# Autodesk Inventor assembly: V1Towers
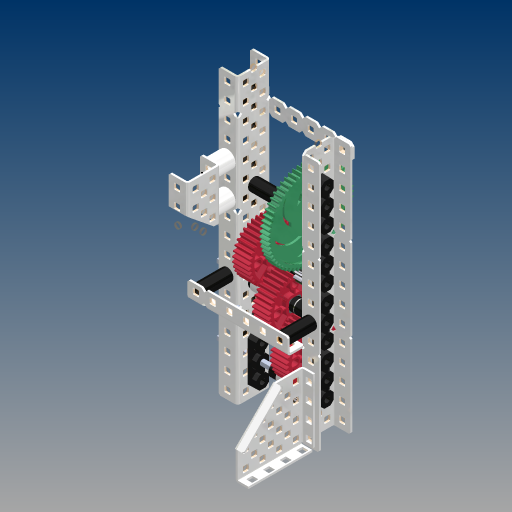
[picture p0: Inventor's stored thumbnail of the model, 512x512]
Saved by Autodesk Inventor 2023 (Build 270158000, 158)
## iProperties
Created: 2023-07-20
Part Number: V1Towers
Document SubType Name: Assembly
Designer: eddie
Author: eddie
## Documents named in this file (26)
- C:\Users\eddie\Documents\81208X-Over-Under-CAD\V1\V1Towers.iam
- C:\Users\eddie\Documents\81208X-Over-Under-CAD\VEX-CAD-Inventor-1.4.0\Structure\C Channel\Aluminum 1x2x1\Alu C 1x2x1x15.ipt
- C:\Users\eddie\Documents\81208X-Over-Under-CAD\VEX-CAD-Inventor-1.4.0\Structure\C Channel\Aluminum 1x2x1\Alu C 1x2x1x17.ipt
- C:\Users\eddie\Documents\81208X-Over-Under-CAD\VEX-CAD-Inventor-1.4.0\Structure\Plate\Aluminum\Alu Plate 1x6.ipt
- C:\Users\eddie\Documents\81208X-Over-Under-CAD\VEX-CAD-Inventor-1.4.0\Motion\Spacers\Spacer Nylon .375 OD\NSpacer .375 OD x .375.ipt
- C:\Users\eddie\Documents\81208X-Over-Under-CAD\VEX-CAD-Inventor-1.4.0\Motion\Spacers\Spacer Nylon .375 OD.ipt
- C:\Users\eddie\Documents\81208X-Over-Under-CAD\VEX-CAD-Inventor-1.4.0\Motion\Spacers\Spacer Nylon .375 OD\NSpacer .375 OD x .500.ipt
- C:\Users\eddie\Documents\81208X-Over-Under-CAD\VEX-CAD-Inventor-1.4.0\Structure\Angle\Aluminum\1x1\Alu Angle 1x1x6.ipt
- C:\Users\eddie\Documents\81208X-Over-Under-CAD\VEX-CAD-Inventor-1.4.0\Motion\Spacers\Spacer Nylon .500 OD\NSpacer White .500 OD x .500.ipt
- C:\Users\eddie\Documents\81208X-Over-Under-CAD\VEX-CAD-Inventor-1.4.0\Motion\Spacers\Spacer Nylon .500 OD.ipt
- C:\Users\eddie\Documents\81208X-Over-Under-CAD\Custom-parts\3x2 channel triangular slice.ipt
- C:\Users\eddie\Documents\81208X-Over-Under-CAD\VEX-CAD-Inventor-1.4.0\Motion\Shaft LS\Bearing Flat.ipt
- C:\Users\eddie\Documents\81208X-Over-Under-CAD\VEX-CAD-Inventor-1.4.0\Structure\Hardware\Nut Alu.ipt
- C:\Users\eddie\Documents\81208X-Over-Under-CAD\VEX-CAD-Inventor-1.4.0\Motion\Gears\HS Gear\HS 12T Gear, Circle.iam
- C:\Users\eddie\Documents\81208X-Over-Under-CAD\VEX-CAD-Inventor-1.4.0\Motion\Gears\HS Gear.iam
- C:\Users\eddie\Documents\81208X-Over-Under-CAD\VEX-CAD-Inventor-1.4.0\Motion\Shaft LS\Shaft LS\Shaft LS 3.0.ipt
- C:\Users\eddie\Documents\81208X-Over-Under-CAD\VEX-CAD-Inventor-1.4.0\Motion\Shaft LS\Shaft LS.ipt
- C:\Users\eddie\Documents\81208X-Over-Under-CAD\Custom-parts\Shaft Collar.ipt
- C:\Users\eddie\Documents\81208X-Over-Under-CAD\VEX-CAD-Inventor-1.4.0\Motion\Gears\LS 12T Gear Steel.ipt
- C:\Users\eddie\Documents\81208X-Over-Under-CAD\VEX-CAD-Inventor-1.4.0\Motion\Spacers\Spacer Nylon .375 OD\NSpacer .375 OD x .125.ipt
- C:\Users\eddie\Documents\81208X-Over-Under-CAD\VEX-CAD-Inventor-1.4.0\Motion\Spacers\Spacer Nylon .375 OD\NSpacer .375 OD x .250.ipt
- C:\Users\eddie\Documents\81208X-Over-Under-CAD\VEX-CAD-Inventor-1.4.0\Motion\Gears\HS Gear\HS 36T Gear, Square.iam
- C:\Users\eddie\Documents\81208X-Over-Under-CAD\VEX-CAD-Inventor-1.4.0\Motion\Spacers\Washer Steel\SWasher .375 OD x .031250.ipt
- C:\Users\eddie\Documents\81208X-Over-Under-CAD\VEX-CAD-Inventor-1.4.0\Motion\Spacers\Washer Steel.ipt
- C:\Users\eddie\Documents\81208X-Over-Under-CAD\VEX-CAD-Inventor-1.4.0\Motion\Gears\LS 60T Gear.ipt
- C:\Users\eddie\Documents\81208X-Over-Under-CAD\Custom-parts\Angle Corner Gusset.ipt
## Components (60 placed, 20 different names)
1. Alu C 1x2x1x15:1 — Insert:1, Insert:3, Insert:11, Insert:12, Insert:13, Insert:14, Insert:19, Insert:26, Insert:32, Insert:39, Insert:46, Insert:53, Insert:59
2. Alu C 1x2x1x17:1 — Insert:2, Insert:5, Insert:8, Insert:9, Insert:15, Insert:16, Insert:17, Insert:18, Insert:31
3. Alu Plate 1x6:1 — Insert:1, Insert:2
4. NSpacer .375 OD x .375:1 — Insert:3, Insert:4
5. NSpacer .375 OD x .500:2 — Insert:4, Insert:7
6. NSpacer .375 OD x .375:3 — Insert:5, Insert:6
7. NSpacer .375 OD x .500:4 — Insert:6
8. Alu Angle 1x1x6:1 — Insert:7
9. NSpacer White .500 OD x .500:1 — Insert:9, Insert:10
10. NSpacer White .500 OD x .500:2 — Insert:8
11. 3x2 channel triangular slice:1 — Insert:10
12. Bearing Flat:1 — Insert:14, Insert:21, Insert:22
13. Bearing Flat:2 — Insert:11, Insert:25
14. Bearing Flat:3 — Insert:13, Insert:23
15. Bearing Flat:4 — Insert:12, Insert:24
16. Bearing Flat:5 — Insert:16
17. Bearing Flat:6 — Insert:15
18. Bearing Flat:7 — Insert:17
19. Bearing Flat:8 — Insert:18
20. Nut Alu:1 — Insert:19, Insert:20
21. HS 12T Gear, Circle:1 [sub-assembly] — Insert:20
22. Shaft LS 3.0:1 — Insert:24
23. Shaft LS 3.0:2 — Insert:25
24. Shaft LS 3.0:3 — Insert:21
25. Shaft LS 3.0:4 — Insert:22
26. Shaft LS 3.0:5 — Insert:23
27. Shaft Collar:1 — Insert:26, Insert:27
28. LS 12T Gear Steel:1 — Insert:27, Insert:28
29. NSpacer .375 OD x .125:5 — Insert:28, Insert:29
30. Shaft Collar:2 — Insert:29, Insert:30
31. NSpacer .375 OD x .250:6 — Insert:30
32. Bearing Flat:9 — Insert:31
33. NSpacer .375 OD x .125:7 — Insert:32, Insert:33
34. HS 36T Gear, Square:2 [sub-assembly] — Insert:33, Insert:34
35. LS 12T Gear Steel:2 — Insert:34, Insert:35
36. NSpacer .375 OD x .375:8 — Insert:35, Insert:36
37. Shaft Collar:3 — Insert:36, Insert:37
38. NSpacer .375 OD x .125:9 — Insert:37, Insert:38
39. NSpacer .375 OD x .125:10 — Insert:38
40. NSpacer .375 OD x .500:11 — Insert:39, Insert:40
41. SWasher .375 OD x .031250:1 — Insert:40, Insert:41
42. NSpacer .375 OD x .125:12 — Insert:41, Insert:42
43. HS 36T Gear, Square:3 [sub-assembly] — Insert:42, Insert:43
44. LS 12T Gear Steel:3 — Insert:43, Insert:44
45. Shaft Collar:4 — Insert:44, Insert:45
46. NSpacer .375 OD x .125:13 — Insert:45
47. NSpacer .375 OD x .125:14 — Insert:46, Insert:47
48. LS 60T Gear:1 — Insert:47, Insert:48
49. Shaft Collar:5 — Insert:48, Insert:49
50. NSpacer .375 OD x .375:15 — Insert:49, Insert:50
51. NSpacer .375 OD x .375:16 — Insert:51, Insert:52
52. NSpacer .375 OD x .250:17 — Insert:50, Insert:51
53. NSpacer .375 OD x .125:18 — Insert:52
54. NSpacer .375 OD x .250:19 — Insert:56, Insert:57
55. NSpacer .375 OD x .125:20 — Insert:53, Insert:54
56. LS 12T Gear Steel:4 — Insert:54, Insert:55
57. NSpacer .375 OD x .500:21 — Insert:55, Insert:56
58. HS 36T Gear, Square:4 [sub-assembly] — Insert:57, Insert:58
59. NSpacer .375 OD x .125:22 — Insert:58
60. Angle Corner Gusset:1 — Insert:59
## Relationships (59: Insert 59)
- Insert:1: Alu C 1x2x1x15:1 ↔ Alu Plate 1x6:1
- Insert:2: Alu C 1x2x1x17:1 ↔ Alu Plate 1x6:1
- Insert:3: Alu C 1x2x1x15:1 ↔ NSpacer .375 OD x .375:1
- Insert:4: NSpacer .375 OD x .375:1 ↔ NSpacer .375 OD x .500:2
- Insert:5: Alu C 1x2x1x17:1 ↔ NSpacer .375 OD x .375:3
- Insert:6: NSpacer .375 OD x .375:3 ↔ NSpacer .375 OD x .500:4
- Insert:7: NSpacer .375 OD x .500:2 ↔ Alu Angle 1x1x6:1
- Insert:8: Alu C 1x2x1x17:1 ↔ NSpacer White .500 OD x .500:2
- Insert:9: Alu C 1x2x1x17:1 ↔ NSpacer White .500 OD x .500:1
- Insert:10: NSpacer White .500 OD x .500:1 ↔ 3x2 channel triangular slice:1
- Insert:11: Alu C 1x2x1x15:1 ↔ Bearing Flat:2
- Insert:12: Alu C 1x2x1x15:1 ↔ Bearing Flat:4
- Insert:13: Alu C 1x2x1x15:1 ↔ Bearing Flat:3
- Insert:14: Alu C 1x2x1x15:1 ↔ Bearing Flat:1
- Insert:15: Alu C 1x2x1x17:1 ↔ Bearing Flat:6
- Insert:16: Alu C 1x2x1x17:1 ↔ Bearing Flat:5
- Insert:17: Alu C 1x2x1x17:1 ↔ Bearing Flat:7
- Insert:18: Alu C 1x2x1x17:1 ↔ Bearing Flat:8
- Insert:19: Alu C 1x2x1x15:1 ↔ Nut Alu:1
- Insert:20: Nut Alu:1 ↔ HS 12T Gear, Circle:1
- Insert:21: Bearing Flat:1 ↔ Shaft LS 3.0:3
- Insert:22: Bearing Flat:1 ↔ Shaft LS 3.0:4
- Insert:23: Bearing Flat:3 ↔ Shaft LS 3.0:5
- Insert:24: Bearing Flat:4 ↔ Shaft LS 3.0:1
- Insert:25: Bearing Flat:2 ↔ Shaft LS 3.0:2
- Insert:26: Alu C 1x2x1x15:1 ↔ Shaft Collar:1
- Insert:27: Shaft Collar:1 ↔ LS 12T Gear Steel:1
- Insert:28: LS 12T Gear Steel:1 ↔ NSpacer .375 OD x .125:5
- Insert:29: NSpacer .375 OD x .125:5 ↔ Shaft Collar:2
- Insert:30: Shaft Collar:2 ↔ NSpacer .375 OD x .250:6
- Insert:31: Alu C 1x2x1x17:1 ↔ Bearing Flat:9
- Insert:32: Alu C 1x2x1x15:1 ↔ NSpacer .375 OD x .125:7
- Insert:33: NSpacer .375 OD x .125:7 ↔ HS 36T Gear, Square:2
- Insert:34: HS 36T Gear, Square:2 ↔ LS 12T Gear Steel:2
- Insert:35: LS 12T Gear Steel:2 ↔ NSpacer .375 OD x .375:8
- Insert:36: NSpacer .375 OD x .375:8 ↔ Shaft Collar:3
- Insert:37: Shaft Collar:3 ↔ NSpacer .375 OD x .125:9
- Insert:38: NSpacer .375 OD x .125:9 ↔ NSpacer .375 OD x .125:10
- Insert:39: Alu C 1x2x1x15:1 ↔ NSpacer .375 OD x .500:11
- Insert:40: NSpacer .375 OD x .500:11 ↔ SWasher .375 OD x .031250:1
- Insert:41: SWasher .375 OD x .031250:1 ↔ NSpacer .375 OD x .125:12
- Insert:42: NSpacer .375 OD x .125:12 ↔ HS 36T Gear, Square:3
- Insert:43: HS 36T Gear, Square:3 ↔ LS 12T Gear Steel:3
- Insert:44: LS 12T Gear Steel:3 ↔ Shaft Collar:4
- Insert:45: Shaft Collar:4 ↔ NSpacer .375 OD x .125:13
- Insert:46: Alu C 1x2x1x15:1 ↔ NSpacer .375 OD x .125:14
- Insert:47: NSpacer .375 OD x .125:14 ↔ LS 60T Gear:1
- Insert:48: LS 60T Gear:1 ↔ Shaft Collar:5
- Insert:49: Shaft Collar:5 ↔ NSpacer .375 OD x .375:15
- Insert:50: NSpacer .375 OD x .375:15 ↔ NSpacer .375 OD x .250:17
- Insert:51: NSpacer .375 OD x .375:16 ↔ NSpacer .375 OD x .250:17
- Insert:52: NSpacer .375 OD x .375:16 ↔ NSpacer .375 OD x .125:18
- Insert:53: Alu C 1x2x1x15:1 ↔ NSpacer .375 OD x .125:20
- Insert:54: NSpacer .375 OD x .125:20 ↔ LS 12T Gear Steel:4
- Insert:55: LS 12T Gear Steel:4 ↔ NSpacer .375 OD x .500:21
- Insert:56: NSpacer .375 OD x .250:19 ↔ NSpacer .375 OD x .500:21
- Insert:57: NSpacer .375 OD x .250:19 ↔ HS 36T Gear, Square:4
- Insert:58: HS 36T Gear, Square:4 ↔ NSpacer .375 OD x .125:22
- Insert:59: Alu C 1x2x1x15:1 ↔ Angle Corner Gusset:1
